# Autodesk Inventor assembly: Main_afterRhino_V2
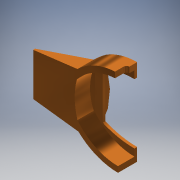
[picture p0: Inventor's stored thumbnail of the model, 180x180]
Saved by Autodesk Inventor 2019 (Build 230136000, 136)
## iProperties
Created: 2021-03-09
Part Number: Main_afterRhino_V2
Material: Generisch
Document SubType Name: Assembly
Designer: Bergi
Author: Bergi
## Documents named in this file (3)
- C:\Users\Bergi\Desktop\3D Sketches\Bulova\Main_afterRhino_V2.iam
- C:\Users\Bergi\Desktop\3D Sketches\Bulova\Main_afterRhino_V2.ipt
- C:\Users\Bergi\Desktop\3D Sketches\Bulova\Main_Rhino_geometry.ipt
## Components (2 placed, 2 different names)
1. Main_afterRhino_V2:1 — Fluchtend:2, Passend:1, Passend:2
2. Main_Rhino_geometry:1 — Fluchtend:2, Passend:1, Passend:2
## Relationships (3: Mate 2, Flush 1)
- Fluchtend:2 [Flush]: Main_afterRhino_V2:1 ↔ Main_Rhino_geometry:1
- Passend:1 [Mate]: Main_afterRhino_V2:1 ↔ Main_Rhino_geometry:1
- Passend:2 [Mate]: Main_afterRhino_V2:1 ↔ Main_Rhino_geometry:1
